# Autodesk Inventor assembly: pcb_assembled
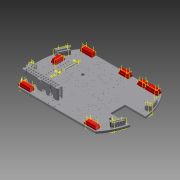
[picture p0: Inventor's stored thumbnail of the model, 180x180]
Saved by Autodesk Inventor 2014 (Build 180170000, 170)
## iProperties
Created: 2013-08-24
Part Number: pcb_assembled
Document SubType Name: Assembly
Designer: Felix
Author: Felix
## Documents named in this file (10)
- C:\Users\Felix\Desktop\Beep\Hardware\3D-CAD\parts\electronic\BEEP\beep_main_assembled.iam
- C:\Users\Felix\Desktop\Beep\Hardware\3D-CAD\parts\electronic\BEEP\Connectors\8526-4500pl-01.ipt
- C:\Users\Felix\Desktop\Beep\Hardware\3D-CAD\parts\electronic\BEEP\beep_main.ipt
- C:\Users\Felix\Desktop\Beep\Hardware\3D-CAD\parts\electronic\BEEP\Connectors\micro-miniature_steckverbinder_a-32-08v-130x0.ipt
- C:\Users\Felix\Desktop\Beep\Hardware\3D-CAD\parts\electronic\BEEP\Connectors\c-215460-8-h-3d.ipt
- C:\Users\Felix\Desktop\Beep\Hardware\3D-CAD\parts\electronic\BEEP\Connectors\micro-miniature_steckverbinder_a-32-04v-130x0.ipt
- C:\Users\Felix\Desktop\Beep\Hardware\3D-CAD\parts\electronic\BEEP\Connectors\micro-miniature_steckverbinder_a-32-06v-130x0.ipt
- C:\Users\Felix\Desktop\Beep\Hardware\3D-CAD\parts\electronic\BEEP\Connectors\micro-miniature_steckverbinder_a-32-10v-130x0.ipt
- C:\Users\Felix\Desktop\Beep\Hardware\3D-CAD\parts\electronic\BEEP\Connectors\12520.ipt
- C:\Users\Felix\Desktop\Beep\Hardware\3D-CAD\parts\electronic\BEEP\Connectors\12521.ipt
## Components (17 placed, 9 different names)
1. beep_main:1 — Passend:4, Passend:5, Passend:6, Passend:10, Tangential:1, Passend:18, Passend:19, Passend:20, Passend:21, Passend:22, Passend:35, Passend:36, Passend:37, Passend:38, Passend:39, Passend:40, Passend:41, Passend:42, Passend:43, Passend:44, Passend:45, Passend:46, Passend:47, Passend:48, Passend:49, Passend:50, Passend:51, Passend:52, Passend:53, Passend:54, Passend:55, Passend:56, Passend:57, Passend:58, Passend:59, Passend:73, Passend:74, Passend:76, Passend:77, Passend:79, Passend:80, Passend:81, Passend:86, Passend:87, Passend:88, Passend:89, Passend:90, Passend:91, Passend:92, Passend:93, Passend:94, Passend:95, Passend:96, Passend:97, Passend:98, Passend:99, Passend:100, Passend:101, Passend:102, Passend:103, Passend:104, Passend:105, Passend:106, Passend:107, Passend:108
2. 8526-4500pl-01:1 — Passend:4, Passend:5, Passend:6
3. micro-miniature_steckverbinder_a-32-08v-130x0:1 — Passend:18, Passend:21, Passend:102, Passend:103, Passend:104
4. micro-miniature_steckverbinder_a-32-08v-130x0:2 — Passend:19, Passend:99, Passend:100, Passend:101
5. micro-miniature_steckverbinder_a-32-08v-130x0:3 — Passend:20, Passend:96, Passend:97, Passend:98
6. micro-miniature_steckverbinder_a-32-08v-130x0:4 — Passend:22, Passend:93, Passend:94, Passend:95
7. c-215460-8-h-3d:1 — Passend:35, Passend:36, Passend:37, Passend:38
8. c-215460-8-h-3d:2 — Passend:40, Passend:48, Passend:49, Passend:50
9. c-215460-8-h-3d:3 — Passend:41, Passend:45, Passend:46, Passend:47
10. c-215460-8-h-3d:4 — Passend:39, Passend:42, Passend:43, Passend:44
11. micro-miniature_steckverbinder_a-32-04v-130x0:1 — Passend:52, Passend:54, Passend:55, Passend:56
12. micro-miniature_steckverbinder_a-32-04v-130x0:2 — Passend:53, Passend:74, Passend:76, Passend:77
13. micro-miniature_steckverbinder_a-32-06v-130x0:1 — Passend:51, Passend:57, Passend:58, Passend:59
14. micro-miniature_steckverbinder_a-32-10v-130x0:1 — Passend:73, Passend:79, Passend:80, Passend:81
15. 12520:1 — Passend:87, Passend:90, Passend:91
16. 12521:1 — Passend:86, Passend:88, Passend:89
17. micro-miniature_steckverbinder_a-32-06v-130x0:2 — Passend:105, Passend:106, Passend:107, Passend:108
## Relationships (65: Mate 64, Tangent 1)
- Passend:4 [Mate]: beep_main:1 ↔ 8526-4500pl-01:1
- Passend:5 [Mate]: beep_main:1 ↔ 8526-4500pl-01:1
- Passend:6 [Mate]: beep_main:1 ↔ 8526-4500pl-01:1
- Passend:10 [Mate]: beep_main:1
- Tangential:1: beep_main:1
- Passend:18 [Mate]: beep_main:1 ↔ micro-miniature_steckverbinder_a-32-08v-130x0:1
- Passend:19 [Mate]: beep_main:1 ↔ micro-miniature_steckverbinder_a-32-08v-130x0:2
- Passend:20 [Mate]: beep_main:1 ↔ micro-miniature_steckverbinder_a-32-08v-130x0:3
- Passend:21 [Mate]: beep_main:1 ↔ micro-miniature_steckverbinder_a-32-08v-130x0:1
- Passend:22 [Mate]: beep_main:1 ↔ micro-miniature_steckverbinder_a-32-08v-130x0:4
- Passend:35 [Mate]: beep_main:1 ↔ c-215460-8-h-3d:1
- Passend:36 [Mate]: beep_main:1 ↔ c-215460-8-h-3d:1
- Passend:37 [Mate]: beep_main:1 ↔ c-215460-8-h-3d:1
- Passend:38 [Mate]: beep_main:1 ↔ c-215460-8-h-3d:1
- Passend:39 [Mate]: beep_main:1 ↔ c-215460-8-h-3d:4
- Passend:40 [Mate]: beep_main:1 ↔ c-215460-8-h-3d:2
- Passend:41 [Mate]: beep_main:1 ↔ c-215460-8-h-3d:3
- Passend:42 [Mate]: beep_main:1 ↔ c-215460-8-h-3d:4
- Passend:43 [Mate]: beep_main:1 ↔ c-215460-8-h-3d:4
- Passend:44 [Mate]: beep_main:1 ↔ c-215460-8-h-3d:4
- Passend:45 [Mate]: beep_main:1 ↔ c-215460-8-h-3d:3
- Passend:46 [Mate]: beep_main:1 ↔ c-215460-8-h-3d:3
- Passend:47 [Mate]: beep_main:1 ↔ c-215460-8-h-3d:3
- Passend:48 [Mate]: beep_main:1 ↔ c-215460-8-h-3d:2
- Passend:49 [Mate]: beep_main:1 ↔ c-215460-8-h-3d:2
- Passend:50 [Mate]: beep_main:1 ↔ c-215460-8-h-3d:2
- Passend:51 [Mate]: beep_main:1 ↔ micro-miniature_steckverbinder_a-32-06v-130x0:1
- Passend:52 [Mate]: beep_main:1 ↔ micro-miniature_steckverbinder_a-32-04v-130x0:1
- Passend:53 [Mate]: beep_main:1 ↔ micro-miniature_steckverbinder_a-32-04v-130x0:2
- Passend:54 [Mate]: beep_main:1 ↔ micro-miniature_steckverbinder_a-32-04v-130x0:1
- Passend:55 [Mate]: beep_main:1 ↔ micro-miniature_steckverbinder_a-32-04v-130x0:1
- Passend:56 [Mate]: beep_main:1 ↔ micro-miniature_steckverbinder_a-32-04v-130x0:1
- Passend:57 [Mate]: beep_main:1 ↔ micro-miniature_steckverbinder_a-32-06v-130x0:1
- Passend:58 [Mate]: beep_main:1 ↔ micro-miniature_steckverbinder_a-32-06v-130x0:1
- Passend:59 [Mate]: beep_main:1 ↔ micro-miniature_steckverbinder_a-32-06v-130x0:1
- Passend:73 [Mate]: beep_main:1 ↔ micro-miniature_steckverbinder_a-32-10v-130x0:1
- Passend:74 [Mate]: beep_main:1 ↔ micro-miniature_steckverbinder_a-32-04v-130x0:2
- Passend:76 [Mate]: beep_main:1 ↔ micro-miniature_steckverbinder_a-32-04v-130x0:2
- Passend:77 [Mate]: beep_main:1 ↔ micro-miniature_steckverbinder_a-32-04v-130x0:2
- Passend:79 [Mate]: beep_main:1 ↔ micro-miniature_steckverbinder_a-32-10v-130x0:1
- Passend:80 [Mate]: beep_main:1 ↔ micro-miniature_steckverbinder_a-32-10v-130x0:1
- Passend:81 [Mate]: beep_main:1 ↔ micro-miniature_steckverbinder_a-32-10v-130x0:1
- Passend:86 [Mate]: beep_main:1 ↔ 12521:1
- Passend:87 [Mate]: beep_main:1 ↔ 12520:1
- Passend:88 [Mate]: beep_main:1 ↔ 12521:1
- Passend:89 [Mate]: beep_main:1 ↔ 12521:1
- Passend:90 [Mate]: beep_main:1 ↔ 12520:1
- Passend:91 [Mate]: beep_main:1 ↔ 12520:1
- Passend:92 [Mate]: beep_main:1
- Passend:93 [Mate]: beep_main:1 ↔ micro-miniature_steckverbinder_a-32-08v-130x0:4
- Passend:94 [Mate]: beep_main:1 ↔ micro-miniature_steckverbinder_a-32-08v-130x0:4
- Passend:95 [Mate]: beep_main:1 ↔ micro-miniature_steckverbinder_a-32-08v-130x0:4
- Passend:96 [Mate]: beep_main:1 ↔ micro-miniature_steckverbinder_a-32-08v-130x0:3
- Passend:97 [Mate]: beep_main:1 ↔ micro-miniature_steckverbinder_a-32-08v-130x0:3
- Passend:98 [Mate]: beep_main:1 ↔ micro-miniature_steckverbinder_a-32-08v-130x0:3
- Passend:99 [Mate]: beep_main:1 ↔ micro-miniature_steckverbinder_a-32-08v-130x0:2
- Passend:100 [Mate]: beep_main:1 ↔ micro-miniature_steckverbinder_a-32-08v-130x0:2
- Passend:101 [Mate]: beep_main:1 ↔ micro-miniature_steckverbinder_a-32-08v-130x0:2
- Passend:102 [Mate]: beep_main:1 ↔ micro-miniature_steckverbinder_a-32-08v-130x0:1
- Passend:103 [Mate]: beep_main:1 ↔ micro-miniature_steckverbinder_a-32-08v-130x0:1
- Passend:104 [Mate]: beep_main:1 ↔ micro-miniature_steckverbinder_a-32-08v-130x0:1
- Passend:105 [Mate]: beep_main:1 ↔ micro-miniature_steckverbinder_a-32-06v-130x0:2
- Passend:106 [Mate]: beep_main:1 ↔ micro-miniature_steckverbinder_a-32-06v-130x0:2
- Passend:107 [Mate]: beep_main:1 ↔ micro-miniature_steckverbinder_a-32-06v-130x0:2
- Passend:108 [Mate]: beep_main:1 ↔ micro-miniature_steckverbinder_a-32-06v-130x0:2
